# Autodesk Inventor assembly: Ensamble chaveta exterior mas tensor polea
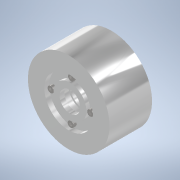
[picture p0: Inventor's stored thumbnail of the model, 180x180]
Saved by Autodesk Inventor 2021 (Build 250183000, 183)
## iProperties
Created: 2021-01-08
Part Number: Ensamble chaveta exterior mas tensor polea
Document SubType Name: Assembly
Designer: dieku
Author: dieku
## Documents named in this file (4)
- C:\Users\dieku\Documents\GitHub\tallerDibujoIngenieria\Ensambles\Ensamble chaveta exterior mas tensor polea.iam
- C:\Users\dieku\Documents\GitHub\tallerDibujoIngenieria\Partes\Cilindro Tensor.ipt
- C:\Users\dieku\Documents\GitHub\tallerDibujoIngenieria\Partes\DIN 912 - M6 x 1 x 16 x 13,5.ipt
- C:\Users\dieku\Documents\GitHub\tallerDibujoIngenieria\Partes\tensorpolea.ipt
## Components (6 placed, 3 different names)
1. Cilindro Tensor:1 — Mate:1, Mate:2, Insert:3, Insert:4, Insert:5
2. DIN 912 - M6 x 1 x 16 x 13,5:3 — Insert:2
3. tensorpolea:1 — Mate:1, Mate:2, Insert:2
4. DIN 912 - M6 x 1 x 16 x 13,5:4 — Insert:5
5. DIN 912 - M6 x 1 x 16 x 13,5:5 — Insert:4
6. DIN 912 - M6 x 1 x 16 x 13,5:6 — Insert:3
## Relationships (6: Insert 4, Mate 2)
- Mate:1: Cilindro Tensor:1 ↔ tensorpolea:1
- Mate:2: Cilindro Tensor:1 ↔ tensorpolea:1
- Insert:2 (-16 mm): DIN 912 - M6 x 1 x 16 x 13,5:3 ↔ tensorpolea:1
- Insert:3 (-15 mm): Cilindro Tensor:1 ↔ DIN 912 - M6 x 1 x 16 x 13,5:6
- Insert:4: Cilindro Tensor:1 ↔ DIN 912 - M6 x 1 x 16 x 13,5:5
- Insert:5: Cilindro Tensor:1 ↔ DIN 912 - M6 x 1 x 16 x 13,5:4
